# Autodesk Inventor assembly: TO-220 Transistor
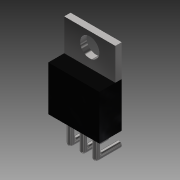
[picture p0: Inventor's stored thumbnail of the model, 180x180]
Saved by Autodesk Inventor 2013 (Build 170138000, 138)
## iProperties
Created: 2014-12-22
Part Number: TO-220 Transistor
Document SubType Name: Assembly
Designer: Kyle
Author: Kyle
## Documents named in this file (4)
- C:\Users\Kyle\Documents\Autodesk\Output\Inventor 2013\Electronics\Transistors\TO-220 Transistor.iam
- C:\Users\Kyle\Documents\Autodesk\Output\Inventor 2013\Electronics\Sub-Components\Multipieces\TO-220 Transistor Body.ipt
- C:\Users\Kyle\Documents\Autodesk\Output\Inventor 2013\Electronics\Sub-Components\Multipieces\TO-220 Transistor Sink.ipt
- C:\Users\Kyle\Documents\Autodesk\Output\Inventor 2013\Electronics\Sub-Components\Leads\TO-220 Transistor Bent Lead.ipt
## Components (5 placed, 3 different names)
1. TO-220 Transistor Body:1 — Mate:1, Flush:1, Flush:2, Mate:2, Angle:1, Mate:3, Mate:4, Angle:2, Mate:5, Mate:6, Angle:3, Mate:7, Mate:10
2. TO-220 Transistor Sink:1 — Mate:1, Flush:1, Flush:2
3. TO-220 Transistor Bent Lead:1 — Mate:4, Angle:2, Mate:5, Mate:8, Mate:10
4. TO-220 Transistor Bent Lead:2 — Mate:6, Angle:3, Mate:7, Mate:9
5. TO-220 Transistor Bent Lead:3 — Mate:2, Angle:1, Mate:3, Mate:8, Mate:9
## Relationships (15: Mate 10, Angle 3, Flush 2)
- Mate:1: TO-220 Transistor Body:1 ↔ TO-220 Transistor Sink:1
- Flush:1: TO-220 Transistor Body:1 ↔ TO-220 Transistor Sink:1
- Flush:2: TO-220 Transistor Body:1 ↔ TO-220 Transistor Sink:1
- Mate:2: TO-220 Transistor Body:1 ↔ TO-220 Transistor Bent Lead:3
- Angle:1 (0 deg): TO-220 Transistor Body:1 ↔ TO-220 Transistor Bent Lead:3
- Mate:3 (-2.54 mm): TO-220 Transistor Body:1 ↔ TO-220 Transistor Bent Lead:3
- Mate:4: TO-220 Transistor Body:1 ↔ TO-220 Transistor Bent Lead:1
- Angle:2 (0 deg): TO-220 Transistor Body:1 ↔ TO-220 Transistor Bent Lead:1
- Mate:5 (-2.54 mm): TO-220 Transistor Body:1 ↔ TO-220 Transistor Bent Lead:1
- Mate:6: TO-220 Transistor Body:1 ↔ TO-220 Transistor Bent Lead:2
- Angle:3 (0 deg): TO-220 Transistor Body:1 ↔ TO-220 Transistor Bent Lead:2
- Mate:7 (-2.54 mm): TO-220 Transistor Body:1 ↔ TO-220 Transistor Bent Lead:2
- Mate:8 (-2.54 mm): TO-220 Transistor Bent Lead:1 ↔ TO-220 Transistor Bent Lead:3
- Mate:9 (2.54 mm): TO-220 Transistor Bent Lead:2 ↔ TO-220 Transistor Bent Lead:3
- Mate:10 (-2.54 mm): TO-220 Transistor Body:1 ↔ TO-220 Transistor Bent Lead:1
